# Autodesk Inventor assembly: WingUnit2L
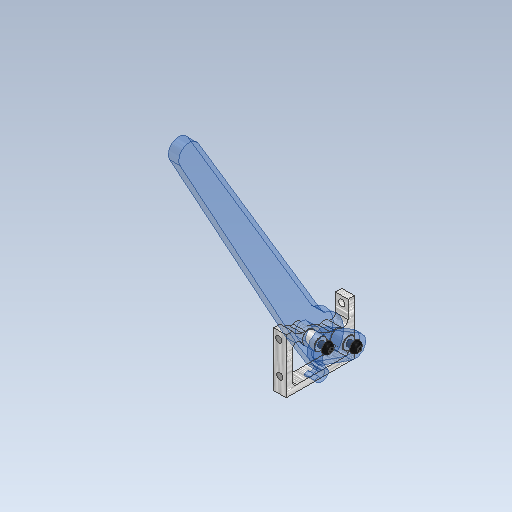
[picture p0: Inventor's stored thumbnail of the model, 512x512]
Saved by Autodesk Inventor 2020.2 (Build 242310000, 310)
## iProperties
Created: 2020-04-23
Part Number: WingUnit2L
Document SubType Name: Assembly
Designer: aoyama
Mass: 19.7102 g
Surface Area: 89.2978 cm^2
Volume: 11.807 cm^3
Density: 1.66937 g/cm^3
Author: aoyama
## Documents named in this file (6)
- C:\Users\aoyam\Desktop\SRDC_local\Inventor\二年機\Geminiβ\翼\WingUnit2L.iam
- C:\Users\aoyam\Desktop\SRDC_local\Inventor\二年機\Geminiβ\翼\Wing2台座.ipt
- C:\Users\aoyam\Desktop\SRDC_local\Inventor\二年機\Geminiβ\翼\Wing2.ipt
- C:\Users\aoyam\Desktop\SRDC_local\Inventor\二年機\Geminiβ\翼\Wing抑え2.ipt
- C:\Users\aoyam\Desktop\SRDC_local\Inventor\二年機\Geminiβ\汎用部品\スペーサー中空M3L6アルミ.ipt
- C:\Users\aoyam\Desktop\SRDC_local\Inventor\二年機\Geminiβ\汎用部品\ネジボタンM3L15.ipt
## Components (7 placed, 5 different names)
1. Wing2台座:1 — 挿入:3, 挿入:4
2. Wing2:1 — 挿入:9
3. Wing抑え2:1 — 挿入:5, 挿入:6, 挿入:7, 挿入:8
4. スペーサー中空M3L6アルミ:1 — 挿入:3, 挿入:5
5. スペーサー中空M3L6アルミ:2 — 挿入:4, 挿入:8, 挿入:9
6. ネジボタンM3L15:1 — 挿入:7
7. ネジボタンM3L15:2 — 挿入:6
## Relationships (7: Insert 7)
- 挿入:3 [Insert]: Wing2台座:1 ↔ スペーサー中空M3L6アルミ:1
- 挿入:4 [Insert]: Wing2台座:1 ↔ スペーサー中空M3L6アルミ:2
- 挿入:5 [Insert]: Wing抑え2:1 ↔ スペーサー中空M3L6アルミ:1
- 挿入:6 [Insert]: Wing抑え2:1 ↔ ネジボタンM3L15:2
- 挿入:7 [Insert]: Wing抑え2:1 ↔ ネジボタンM3L15:1
- 挿入:8 [Insert]: Wing抑え2:1 ↔ スペーサー中空M3L6アルミ:2
- 挿入:9 [Insert]: Wing2:1 ↔ スペーサー中空M3L6アルミ:2
